# Autodesk Inventor assembly: main
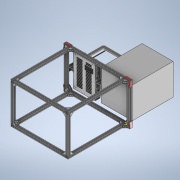
[picture p0: Inventor's stored thumbnail of the model, 180x180]
Saved by Autodesk Inventor 2022 (Build 260153000, 153)
## iProperties
Created: 2022-06-19
Part Number: main
Document SubType Name: Assembly
Designer: logic
Author: logic
## Documents named in this file (10)
- C:\Users\logic\Desktop\3030-profile-frame\main.iam
- C:\Users\logic\Desktop\3030-profile-frame\parts\3030_700.ipt
- C:\Users\logic\Desktop\3030-profile-frame\parts\3030_440.ipt
- C:\Users\logic\Desktop\3030-profile-frame\parts\3030_640.ipt
- C:\Users\logic\Desktop\3030-profile-frame\parts\3030_800.ipt
- C:\Users\logic\Desktop\3030-profile-frame\parts\3030_angle.ipt
- C:\Users\logic\Desktop\3030-profile-frame\parts\top_cover.ipt
- C:\Users\logic\Desktop\3030-profile-frame\parts\top_cover_alt.ipt
- C:\Users\logic\Desktop\3030-profile-frame\parts\Anycubii3Mega Version 2 v4\Anycubii3Mega Version 2.iam
- C:\Users\logic\Desktop\3030-profile-frame\parts\voron.ipt
## Components (42 placed, 9 different names)
1. 3030_700:1 — Flush:7, Mate:4, Flush:8, Flush:9, Flush:10, Mate:5, Mate:30, Flush:32, Mate:33, Mate:50, Mate:53
2. 3030_700:2 — Flush:13, Flush:14, Flush:15, Mate:7, Flush:16, Mate:8, Mate:14, Mate:17, Mate:43, Flush:40, Mate:46
3. 3030_700:3 — Flush:1, Flush:2, Mate:1, Flush:5, Flush:6, Mate:3, Mate:25, Flush:29, Mate:27, Flush:30, Flush:46, Mate:56, Mate:58
4. 3030_700:4 — Mate:2, Flush:3, Flush:4, Flush:21, Mate:11, Flush:22, Mate:18, Flush:26, Flush:27, Mate:20, Flush:36, Mate:38, Mate:41, Flush:37
5. 3030_440:1 — Flush:14, Flush:16, Mate:8, Mate:13, Mate:16, Flush:25, Mate:19, Mate:23, Flush:28
6. 3030_440:2 — Flush:5, Flush:6, Mate:3, Flush:7, Mate:4, Flush:8, Mate:26, Mate:29, Flush:31, Mate:32, Flush:33, Mate:34, Flush:34
7. 3030_440:3 — Flush:11, Flush:12, Mate:6, Flush:17, Flush:18, Mate:9, Mate:49, Flush:44, Mate:54, Mate:63, Mate:69, Mate:70
8. 3030_440:4 — Flush:19, Flush:20, Mate:10, Flush:35, Mate:37, Flush:39, Mate:45, Mate:60, Mate:61, Mate:66, Mate:67
9. 3030_640:1 — Flush:1, Flush:2, Mate:1, Mate:2, Flush:3, Flush:4, Mate:21, Mate:22, Mate:24, Mate:28
10. 3030_640:2 — Flush:9, Flush:10, Mate:5, Flush:13, Flush:15, Mate:7, Mate:12, Flush:23, Flush:24, Mate:15, Mate:31, Mate:35
11. 3030_800:1 — Flush:17, Flush:18, Mate:9, Flush:19, Flush:20, Mate:10, Flush:21, Mate:11, Flush:22, Mate:36, Mate:39, Mate:40, Mate:55, Flush:45, Mate:57, Mate:59, Mate:62, Mate:71
12. 3030_800:2 — Flush:11, Flush:12, Mate:6, Flush:38, Mate:42, Mate:44, Mate:47, Flush:41, Mate:48, Mate:51, Flush:42, Flush:43, Mate:52, Mate:64, Mate:65, Mate:68
13. 3030_angle:1 — Mate:34, Mate:35, Flush:34
14. 3030_angle:2 — Mate:18, Mate:19, Flush:26
15. 3030_angle:3 — Mate:22, Mate:23, Flush:28
16. 3030_angle:4 — Mate:12, Mate:13, Flush:23
17. 3030_angle:5 — Mate:16, Flush:25, Mate:17
18. 3030_angle:6 — Flush:24, Mate:14, Mate:15
19. 3030_angle:7 — Mate:32, Mate:33, Flush:33
20. 3030_angle:8 — Flush:27, Mate:20, Mate:21
21. 3030_angle:9 — Mate:30, Mate:31, Flush:32
22. 3030_angle:10 — Mate:28, Mate:29, Flush:31
23. 3030_angle:11 — Mate:24, Mate:25, Flush:29
24. 3030_angle:12 — Mate:26, Mate:27, Flush:30
25. 3030_angle:13 — Flush:45, Mate:56, Mate:57
26. 3030_angle:14 — Flush:38, Mate:42, Mate:43
27. 3030_angle:15 — Flush:43, Mate:52, Mate:53
28. 3030_angle:16 — Flush:36, Mate:38, Mate:39
29. 3030_angle:17 — Mate:40, Mate:41, Flush:37
30. 3030_angle:18 — Flush:35, Mate:36, Mate:37
31. 3030_angle:19 — Flush:40, Mate:46, Mate:47
32. 3030_angle:20 — Flush:39, Mate:44, Mate:45
33. 3030_angle:21 — Mate:50, Mate:51, Flush:42
34. 3030_angle:22 — Flush:41, Mate:48, Mate:49
35. 3030_angle:23 — Flush:46, Mate:58, Mate:59
36. 3030_angle:24 — Flush:44, Mate:54, Mate:55
37. top_cover:1 — Mate:60, Mate:61, Mate:62
38. top_cover:2 — Mate:63, Mate:64, Mate:65
39. top_cover_alt:1 — Mate:69, Mate:70, Mate:71
40. top_cover_alt:2 — Mate:66, Mate:67, Mate:68
41. Anycubii3Mega Version 2:1 [sub-assembly]
42. voron:1
## Relationships (117: Mate 71, Flush 46)
- Flush:1: 3030_700:3 ↔ 3030_640:1
- Flush:2: 3030_700:3 ↔ 3030_640:1
- Mate:1: 3030_700:3 ↔ 3030_640:1
- Mate:2: 3030_700:4 ↔ 3030_640:1
- Flush:3: 3030_700:4 ↔ 3030_640:1
- Flush:4: 3030_700:4 ↔ 3030_640:1
- Flush:5: 3030_700:3 ↔ 3030_440:2
- Flush:6: 3030_700:3 ↔ 3030_440:2
- Mate:3: 3030_700:3 ↔ 3030_440:2
- Flush:7: 3030_700:1 ↔ 3030_440:2
- Mate:4: 3030_700:1 ↔ 3030_440:2
- Flush:8: 3030_700:1 ↔ 3030_440:2
- Flush:9: 3030_700:1 ↔ 3030_640:2
- Flush:10: 3030_700:1 ↔ 3030_640:2
- Mate:5: 3030_700:1 ↔ 3030_640:2
- Flush:11: 3030_440:3 ↔ 3030_800:2
- Flush:12: 3030_440:3 ↔ 3030_800:2
- Mate:6: 3030_440:3 ↔ 3030_800:2
- Flush:13: 3030_700:2 ↔ 3030_640:2
- Flush:14: 3030_700:2 ↔ 3030_440:1
- Flush:15: 3030_700:2 ↔ 3030_640:2
- Mate:7: 3030_700:2 ↔ 3030_640:2
- Flush:16: 3030_700:2 ↔ 3030_440:1
- Mate:8: 3030_700:2 ↔ 3030_440:1
- Flush:17: 3030_440:3 ↔ 3030_800:1
- Flush:18: 3030_440:3 ↔ 3030_800:1
- Mate:9: 3030_440:3 ↔ 3030_800:1
- Flush:19: 3030_440:4 ↔ 3030_800:1
- Flush:20: 3030_440:4 ↔ 3030_800:1
- Mate:10: 3030_440:4 ↔ 3030_800:1
- Flush:21: 3030_700:4 ↔ 3030_800:1
- Mate:11: 3030_700:4 ↔ 3030_800:1
- Flush:22 (-50 mm): 3030_700:4 ↔ 3030_800:1
- Mate:12: 3030_640:2 ↔ 3030_angle:4
- Mate:13: 3030_440:1 ↔ 3030_angle:4
- Flush:23: 3030_640:2 ↔ 3030_angle:4
- Flush:24: 3030_640:2 ↔ 3030_angle:6
- Mate:14: 3030_700:2 ↔ 3030_angle:6
- Mate:15: 3030_640:2 ↔ 3030_angle:6
- Mate:16: 3030_440:1 ↔ 3030_angle:5
- Flush:25: 3030_440:1 ↔ 3030_angle:5
- Mate:17: 3030_700:2 ↔ 3030_angle:5
- Mate:18: 3030_700:4 ↔ 3030_angle:2
- Mate:19: 3030_440:1 ↔ 3030_angle:2
- Flush:26: 3030_700:4 ↔ 3030_angle:2
- Flush:27: 3030_700:4 ↔ 3030_angle:8
- Mate:20: 3030_700:4 ↔ 3030_angle:8
- Mate:21: 3030_640:1 ↔ 3030_angle:8
- Mate:22: 3030_640:1 ↔ 3030_angle:3
- Mate:23: 3030_440:1 ↔ 3030_angle:3
- Flush:28: 3030_440:1 ↔ 3030_angle:3
- Mate:24: 3030_640:1 ↔ 3030_angle:11
- Mate:25: 3030_700:3 ↔ 3030_angle:11
- Flush:29: 3030_700:3 ↔ 3030_angle:11
- Mate:26: 3030_440:2 ↔ 3030_angle:12
- Mate:27: 3030_700:3 ↔ 3030_angle:12
- Flush:30: 3030_700:3 ↔ 3030_angle:12
- Mate:28: 3030_640:1 ↔ 3030_angle:10
- Mate:29: 3030_440:2 ↔ 3030_angle:10
- Flush:31: 3030_440:2 ↔ 3030_angle:10
- Mate:30: 3030_700:1 ↔ 3030_angle:9
- Mate:31: 3030_640:2 ↔ 3030_angle:9
- Flush:32: 3030_700:1 ↔ 3030_angle:9
- Mate:32: 3030_440:2 ↔ 3030_angle:7
- Mate:33: 3030_700:1 ↔ 3030_angle:7
- Flush:33: 3030_440:2 ↔ 3030_angle:7
- Mate:34: 3030_440:2 ↔ 3030_angle:1
- Mate:35: 3030_640:2 ↔ 3030_angle:1
- Flush:34: 3030_440:2 ↔ 3030_angle:1
- Flush:35: 3030_440:4 ↔ 3030_angle:18
- Mate:36: 3030_800:1 ↔ 3030_angle:18
- Mate:37: 3030_440:4 ↔ 3030_angle:18
- Flush:36: 3030_700:4 ↔ 3030_angle:16
- Mate:38: 3030_700:4 ↔ 3030_angle:16
- Mate:39: 3030_800:1 ↔ 3030_angle:16
- Mate:40: 3030_800:1 ↔ 3030_angle:17
- Mate:41: 3030_700:4 ↔ 3030_angle:17
- Flush:37: 3030_700:4 ↔ 3030_angle:17
- Flush:38: 3030_800:2 ↔ 3030_angle:14
- Mate:42: 3030_800:2 ↔ 3030_angle:14
- Mate:43: 3030_700:2 ↔ 3030_angle:14
- Flush:39: 3030_440:4 ↔ 3030_angle:20
- Mate:44: 3030_800:2 ↔ 3030_angle:20
- Mate:45: 3030_440:4 ↔ 3030_angle:20
- Flush:40: 3030_700:2 ↔ 3030_angle:19
- Mate:46: 3030_700:2 ↔ 3030_angle:19
- Mate:47: 3030_800:2 ↔ 3030_angle:19
- Flush:41: 3030_800:2 ↔ 3030_angle:22
- Mate:48: 3030_800:2 ↔ 3030_angle:22
- Mate:49: 3030_440:3 ↔ 3030_angle:22
- Mate:50: 3030_700:1 ↔ 3030_angle:21
- Mate:51: 3030_800:2 ↔ 3030_angle:21
- Flush:42: 3030_800:2 ↔ 3030_angle:21
- Flush:43: 3030_800:2 ↔ 3030_angle:15
- Mate:52: 3030_800:2 ↔ 3030_angle:15
- Mate:53: 3030_700:1 ↔ 3030_angle:15
- Flush:44: 3030_440:3 ↔ 3030_angle:24
- Mate:54: 3030_440:3 ↔ 3030_angle:24
- Mate:55: 3030_800:1 ↔ 3030_angle:24
- Flush:45: 3030_800:1 ↔ 3030_angle:13
- Flush:46: 3030_700:3 ↔ 3030_angle:23
- Mate:56: 3030_700:3 ↔ 3030_angle:13
- Mate:57: 3030_800:1 ↔ 3030_angle:13
- Mate:58: 3030_700:3 ↔ 3030_angle:23
- Mate:59: 3030_800:1 ↔ 3030_angle:23
- Mate:60: 3030_440:4 ↔ top_cover:1
- Mate:61: 3030_440:4 ↔ top_cover:1
- Mate:62: 3030_800:1 ↔ top_cover:1
- Mate:63: 3030_440:3 ↔ top_cover:2
- Mate:64: 3030_800:2 ↔ top_cover:2
- Mate:65: 3030_800:2 ↔ top_cover:2
- Mate:66: 3030_440:4 ↔ top_cover_alt:2
- Mate:67: 3030_440:4 ↔ top_cover_alt:2
- Mate:68: 3030_800:2 ↔ top_cover_alt:2
- Mate:69: 3030_440:3 ↔ top_cover_alt:1
- Mate:70: 3030_440:3 ↔ top_cover_alt:1
- Mate:71: 3030_800:1 ↔ top_cover_alt:1
